# Autodesk Inventor assembly: LegGroinUnitBasis
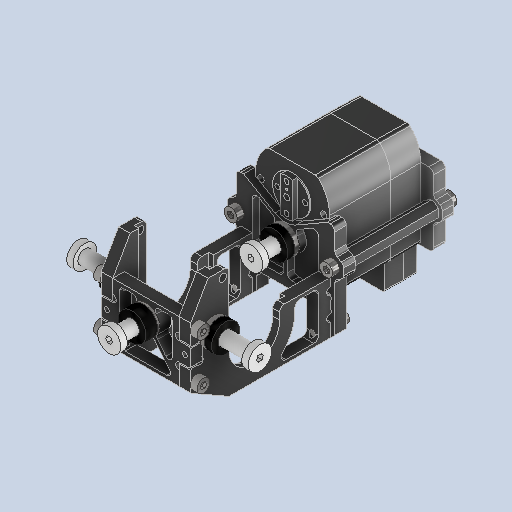
[picture p0: Inventor's stored thumbnail of the model, 512x512]
Saved by Autodesk Inventor 2024.2 (Build 282272000, 272)
## iProperties
Created: 2024-01-08
Part Number: LegGroinUnitBasis
Document SubType Name: Assembly
Designer: Masato Kubotera
Mass: 210.334 g
Surface Area: 373.811 cm^2
Volume: 86.5368 cm^3
Density: 2.43058 g/cm^3
Author: Masato Kubotera
## Documents named in this file (10)
- C:\Users\masato\OneDrive - Chiba Institute of Technology\CIT Brains\RoboCup2024\Mechanic\SUSTAINA-OP2\NativeFiles\Boby\LowerLimb\Legs\LegBases\LegGroinUnitBasis.iam
- C:\Users\masato\OneDrive - Chiba Institute of Technology\CIT Brains\RoboCup2024\Mechanic\SUSTAINA-OP2\NativeFiles\Boby\COTS\Screws\CapScrew\FC-2620EB.ipt
- C:\Users\masato\OneDrive - Chiba Institute of Technology\CIT Brains\RoboCup2024\Mechanic\SUSTAINA-OP2\NativeFiles\Boby\LowerLimb\Legs\LegBases\LegBaseUnitBasis.iam
- C:\Users\masato\OneDrive - Chiba Institute of Technology\CIT Brains\RoboCup2024\Mechanic\SUSTAINA-OP2\NativeFiles\Boby\COTS\Washers\Metal\UUW-0412-10H.ipt
- C:\Users\masato\OneDrive - Chiba Institute of Technology\CIT Brains\RoboCup2024\Mechanic\SUSTAINA-OP2\NativeFiles\Boby\COTS\Washers\Resin\CC-0612-50B.ipt
- C:\Users\masato\OneDrive - Chiba Institute of Technology\CIT Brains\RoboCup2024\Mechanic\SUSTAINA-OP2\NativeFiles\Boby\COTS\Screws\ScrewsWithShoulder\DBTSY4-12-6-DHC.ipt
- C:\Users\masato\OneDrive - Chiba Institute of Technology\CIT Brains\RoboCup2024\Mechanic\SUSTAINA-OP2\NativeFiles\Boby\COTS\Actuators\PMX-SCR-9203HV.ipt
- C:\Users\masato\OneDrive - Chiba Institute of Technology\CIT Brains\RoboCup2024\Mechanic\SUSTAINA-OP2\NativeFiles\Boby\LowerLimb\Legs\LegBases\LegBaseBackFrame.ipt
- C:\Users\masato\OneDrive - Chiba Institute of Technology\CIT Brains\RoboCup2024\Mechanic\SUSTAINA-OP2\NativeFiles\Boby\COTS\Spacers\ABLSBF6-39_5-M3-N3.ipt
- C:\Users\masato\OneDrive - Chiba Institute of Technology\CIT Brains\RoboCup2024\Mechanic\SUSTAINA-OP2\NativeFiles\Boby\COTS\Screws\CapScrew\UC-0310.ipt
## Components (12 placed, 9 different names)
1. LegBaseUnitBasis:1 [sub-assembly] — Flush:1, Mate:3, Mate:4, Insert:8, Insert:18, Insert:19
2. LegBaseBackFrame:1
3. PMX-SCR-9203HV:1
4. UC-0310:1
5. UC-0310:2
6. FC-2620EB:2
7. FC-2620EB:3
8. DBTSY4-12-6-DHC:1
9. ABLSBF6-39_5-M3-N3:1 — Insert:19, Angle:1
10. ABLSBF6-39_5-M3-N3:2 — Insert:18, Angle:2
11. CC-0612-50B:1 — Insert:9
12. UUW-0412-10H:1 — Insert:8, Insert:9
## Relationships (18: Insert 13, Mate 2, Angle 2, Flush 1)
- Flush:1: LegBaseUnitBasis:1
- Mate:3: LegBaseUnitBasis:1
- Mate:4: LegBaseUnitBasis:1
- [Insert]: DBTSY4-12-6-DHC:1 ↔ UUW-0412-10H:1
- Insert:8: LegBaseUnitBasis:1 ↔ UUW-0412-10H:1
- Insert:9: CC-0612-50B:1 ↔ UUW-0412-10H:1
- [Insert]: LegBaseBackFrame:1 ↔ PMX-SCR-9203HV:1
- [Insert]: LegBaseBackFrame:1 ↔ PMX-SCR-9203HV:1
- [Insert]: LegBaseBackFrame:1 ↔ FC-2620EB:2
- [Insert]: LegBaseBackFrame:1 ↔ FC-2620EB:3
- [Insert]: LegBaseBackFrame:1 ↔ ABLSBF6-39_5-M3-N3:1
- [Insert]: LegBaseBackFrame:1 ↔ ABLSBF6-39_5-M3-N3:2
- [Insert]: LegBaseBackFrame:1 ↔ UC-0310:1
- [Insert]: LegBaseBackFrame:1 ↔ UC-0310:2
- Insert:18: LegBaseUnitBasis:1 ↔ ABLSBF6-39_5-M3-N3:2
- Insert:19: LegBaseUnitBasis:1 ↔ ABLSBF6-39_5-M3-N3:1
- Angle:1 (0 deg): ABLSBF6-39_5-M3-N3:1
- Angle:2 (0 deg): ABLSBF6-39_5-M3-N3:2
## Named parameters: d64_d62 = 0 mm, d67_d57 = 0 mm, d69_d59 = 0 mm, d70_d60 = 0 mm
